# Autodesk Inventor assembly: ExcavatorAssembly
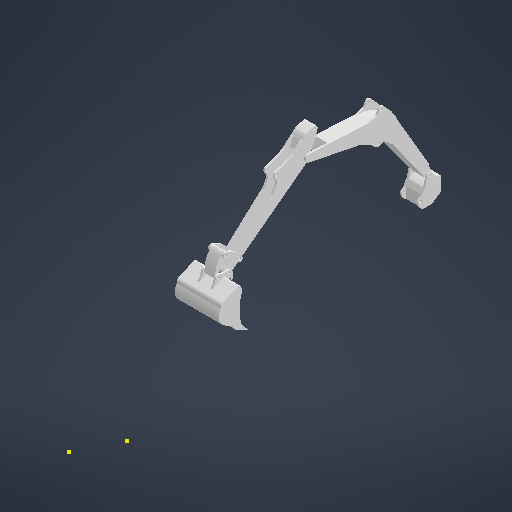
[picture p0: Inventor's stored thumbnail of the model, 512x512]
Saved by Autodesk Inventor 2026 (Build 300175000, 175)
## iProperties
Created: 2025-04-29
Part Number: ExcavatorAssembly
Document SubType Name: Assembly
Designer: elias
Author: elias
## Documents named in this file (7)
- C:\Users\elias\OneDrive\Mechatronics Master 1st\P3-P4\P4\MF2121 - Capstone Course\CAD\ExcavatorAssembly.iam
- C:\Users\elias\OneDrive\Mechatronics Master 1st\P3-P4\P4\MF2121 - Capstone Course\CAD\bas.ipt
- C:\Users\elias\OneDrive\Mechatronics Master 1st\P3-P4\P4\MF2121 - Capstone Course\CAD\bom.ipt
- C:\Users\elias\OneDrive\Mechatronics Master 1st\P3-P4\P4\MF2121 - Capstone Course\CAD\Sticka.ipt
- C:\Users\elias\OneDrive\Mechatronics Master 1st\P3-P4\P4\MF2121 - Capstone Course\CAD\Lankarm_lång.ipt
- C:\Users\elias\OneDrive\Mechatronics Master 1st\P3-P4\P4\MF2121 - Capstone Course\CAD\Lankarm_kort.ipt
- C:\Users\elias\OneDrive\Mechatronics Master 1st\P3-P4\P4\MF2121 - Capstone Course\CAD\Skopa.ipt
## Components (7 placed, 6 different names)
1. bas:1 — Insert:9
2. bom:1 — Insert:2, Insert:9
3. Sticka:1 — Insert:2, Insert:3, Insert:5, Insert:7
4. Lankarm_lång:1 — Insert:4, Insert:6, Insert:8
5. Lankarm_kort:1 — Insert:3, Insert:4
6. Lankarm_kort:2 — Insert:5, Insert:6
7. Skopa:1 — Insert:7, Insert:8
## Relationships (8: Insert 8)
- Insert:2 (25 mm): bom:1 ↔ Sticka:1
- Insert:3: Sticka:1 ↔ Lankarm_kort:1
- Insert:4: Lankarm_lång:1 ↔ Lankarm_kort:1
- Insert:5: Sticka:1 ↔ Lankarm_kort:2
- Insert:6: Lankarm_lång:1 ↔ Lankarm_kort:2
- Insert:7: Sticka:1 ↔ Skopa:1
- Insert:8: Lankarm_lång:1 ↔ Skopa:1
- Insert:9: bas:1 ↔ bom:1
